# Autodesk Inventor assembly: gear_test
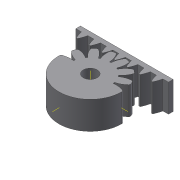
[picture p0: Inventor's stored thumbnail of the model, 180x180]
Saved by Autodesk Inventor 2014 (Build 180170000, 170)
## iProperties
Created: 2015-05-16
Part Number: gear_test
Document SubType Name: Assembly
Designer: Martin
Author: Martin
## Documents named in this file (3)
- C:\Users\Martin\Dropbox\biohand-mec\biohand_v1\fingers\thumb\gear_test.iam
- C:\Users\Martin\Dropbox\biohand-mec\biohand_v1\fingers\thumb\thumb_base.ipt
- C:\Users\Martin\Dropbox\biohand-mec\biohand_v1\fingers\thumb\rack_test.ipt
## Components (2 placed, 2 different names)
1. thumb_base:1 — Mate:1, Mate:2, Flush:1
2. rack_test:1 — Flush:2
## Relationships (4: Mate 2, Flush 2)
- Mate:1: thumb_base:1
- Mate:2: thumb_base:1
- Flush:1: thumb_base:1
- Flush:2: rack_test:1
